# Autodesk Inventor assembly: Idle Bearing Mount
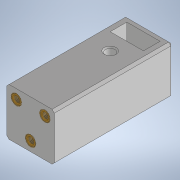
[picture p0: Inventor's stored thumbnail of the model, 180x180]
Saved by Autodesk Inventor 2022 (Build 260153000, 153)
## iProperties
Created: 2022-04-24
Part Number: Idle Bearing Mount
Document SubType Name: Assembly
Designer: Nick
Author: Nick
## Documents named in this file (3)
- Y:\Projects\Mini_Sand_Table\Idle Bearing Mount.iam
- Y:\Projects\Mini_Sand_Table\Idle Bearing Mount.ipt
- Y:\Projects\Mini_Sand_Table\M3 Heat Set Inserts.ipt
## Components (4 placed, 2 different names)
1. Idle Bearing Mount:1 — Insert:1, Insert:2, Insert:3
2. M3 Heat Set Inserts:1 — Insert:1
3. M3 Heat Set Inserts:2 — Insert:2
4. M3 Heat Set Inserts:3 — Insert:3
## Relationships (3: Insert 3)
- Insert:1: Idle Bearing Mount:1 ↔ M3 Heat Set Inserts:1
- Insert:2: Idle Bearing Mount:1 ↔ M3 Heat Set Inserts:2
- Insert:3: Idle Bearing Mount:1 ↔ M3 Heat Set Inserts:3
